# Autodesk Inventor assembly: sle monitoring wrist watch
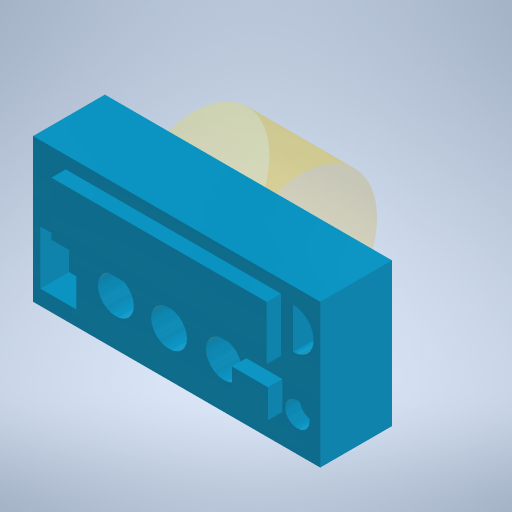
[picture p0: Inventor's stored thumbnail of the model, 512x512]
Saved by Autodesk Inventor 2024 (Build 280153000, 153)
## iProperties
Created: 2024-07-22
Part Number: sle monitoring wrist watch
Document SubType Name: Assembly
Designer: NICODEMUS
Author: NICODEMUS
## Documents named in this file (3)
- C:\Users\NICODEMUS\OneDrive\Dokumente\sle monitoring wrist watch.iam
- C:\Users\NICODEMUS\OneDrive\Dokumente\sle watch.ipt
- C:\Users\NICODEMUS\OneDrive\Dokumente\wrist band.ipt
## Components (2 placed, 2 different names)
1. sle watch:1 — Mate:1
2. wrist band:1 — Mate:1
## Relationships (1: Mate 1)
- Mate:1: sle watch:1 ↔ wrist band:1
